# Autodesk Inventor assembly: ProbeHead V3 - Assembly
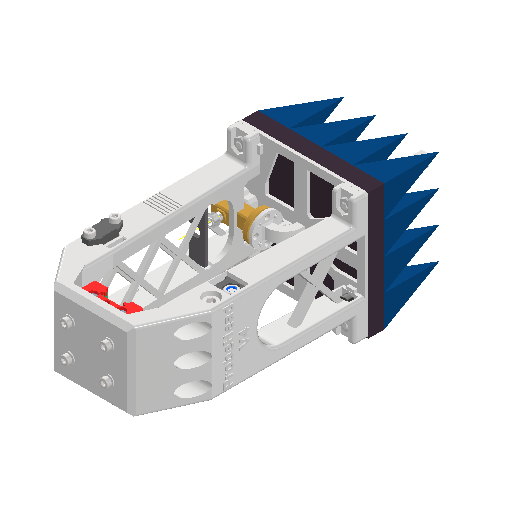
[picture p0: Inventor's stored thumbnail of the model, 512x512]
Saved by Autodesk Inventor 2023.2 (Build 272271000, 271)
## iProperties
Created: 2024-02-09
Part Number: ProbeHead V3 - Assembly
Document SubType Name: Assembly
Designer: Nils Bade
Author: Nils Bade
## Documents named in this file (17)
- C:\Users\nilsb\Documents\Inventor\Projektarbeit-Bade\RatRig_modified\ProbeHead\ProbeHead V4 - Assembly.iam
- C:\Users\nilsb\Documents\Inventor\Projektarbeit-Bade\RatRig_modified\MGN15 Linear-Rail-Block.ipt
- C:\Users\nilsb\Documents\Inventor\Projektarbeit-Bade\RatRig_Standards\face_belt_grabber v2.ipt
- C:\Users\nilsb\Documents\Inventor\Projektarbeit-Bade\Schrauben\Cap Head Screw M3x12 v2.ipt
- C:\Users\nilsb\Documents\Inventor\Projektarbeit-Bade\RatRig_Standards\Hex Nut - M3 v2.ipt
- C:\Users\nilsb\Documents\Inventor\Projektarbeit-Bade\Schrauben\Cap Head Screw M5x40 v2.ipt
- C:\Users\nilsb\Documents\Inventor\Projektarbeit-Bade\RatRig_Standards\Hex Locking Nut - M5 v2.ipt
- C:\Users\nilsb\Documents\Inventor\Projektarbeit-Bade\Schrauben\Washer Simple M3 - DIN6902.ipt
- C:\Users\nilsb\Documents\Inventor\Projektarbeit-Bade\RatRig_modified\ProbeHead\Wire2Probe_Eravant_SWC-15VF-R1-V.ipt
- C:\Users\nilsb\Documents\Inventor\Projektarbeit-Bade\Enclosure\Absorber\Absorber - IHF-Mini.ipt
- C:\Users\nilsb\Documents\Inventor\Projektarbeit-Bade\RatRig_modified\core_xy_belt_grabber_Bade.ipt
- C:\Users\nilsb\Documents\Inventor\Projektarbeit-Bade\RatRig_modified\ProbeHead\ProbeHead_Kabelfixieung_V1.ipt
- C:\Users\nilsb\Documents\Inventor\Projektarbeit-Bade\Enclosure\Magnet-RatrigEnclosure.ipt
- C:\Users\nilsb\Documents\Inventor\Projektarbeit-Bade\RatRig_Standards\Hex Nut - M4 DIN934.ipt
- C:\Users\nilsb\Documents\Inventor\Projektarbeit-Bade\Schrauben\Cap Head Screw M4x8 - DIN912.ipt
- C:\Users\nilsb\Documents\Inventor\Projektarbeit-Bade\RatRig_modified\ProbeHead\ProbeHead-Arms V4.ipt
- C:\Users\nilsb\Documents\Inventor\Projektarbeit-Bade\RatRig_modified\ProbeHead\ProbeAntennas\ProbeAntenna_V1_Long.ipt
## Components (58 placed, 16 different names)
1. ProbeHead-Arms_V4:1 — Passend:96, Passend:97
2. core_xy_belt_grabber_Bade:2
3. core_xy_belt_grabber_Bade:1
4. MGN15 Linear-Rail-Block:1
5. face_belt_grabber v2:1 — Passend:16, Passend:17, Passend:18, Passend:19
6. face_belt_grabber v2:2 — Passend:12, Passend:13, Passend:14, Passend:15
7. Cap Head Screw M3x12 v2:1 — Passend:16, Passend:18, Passend:20
8. Cap Head Screw M3x12 v2:2 — Passend:17, Passend:19, Passend:21
9. Cap Head Screw M3x12 v2:3 — Passend:12, Passend:14, Passend:22
10. Cap Head Screw M3x12 v2:4 — Passend:13, Passend:15, Passend:23
11. Hex Nut - M3 v2:1 — Passend:20
12. Hex Nut - M3 v2:2 — Passend:23
13. Hex Nut - M3 v2:3 — Passend:22
14. Hex Nut - M3 v2:4 — Passend:21
15. Cap Head Screw M5x40 v2:1 — Passend:34
16. Cap Head Screw M5x40 v2:2
17. Hex Locking Nut - M5 v2:1
18. Hex Locking Nut - M5 v2:2 — Passend:34
19. Washer Simple M3 - DIN6902:1 — Passend:59
20. Washer Simple M3 - DIN6902:2 — Passend:56
21. Washer Simple M3 - DIN6902:3 — Passend:58
22. Washer Simple M3 - DIN6902:4 — Passend:57
23. Cap Head Screw M3x12 v2:5 — Passend:59
24. Cap Head Screw M3x12 v2:6 — Passend:58
25. Cap Head Screw M3x12 v2:7 — Passend:56
26. Cap Head Screw M3x12 v2:8 — Passend:57
27. Wire2Probe_Eravant_SWC-15VF-R1-V:1 — Passend:68
28. ProbeAntenna V1 Long:1
29. ProbeHead_Kabelfixieung_V1:1 — Passend:68
30. Magnet-RatrigEnclosure:1
31. Magnet-RatrigEnclosure:2
32. Magnet-RatrigEnclosure:3
33. Magnet-RatrigEnclosure:4
34. Magnet-RatrigEnclosure:5
35. Hex Nut - M4 DIN934:1 — Passend:101
36. Hex Nut - M4 DIN934:2 — Passend:98
37. Hex Nut - M4 DIN934:3 — Passend:99
38. Hex Nut - M4 DIN934:4 — Passend:100
39. Cap Head Screw M4x8 - DIN912:1 — Passend:99
40. Cap Head Screw M4x8 - DIN912:2 — Passend:97, Passend:98
41. Cap Head Screw M4x8 - DIN912:3 — Passend:101
42. Cap Head Screw M4x8 - DIN912:4 — Passend:96, Passend:100
43. Absorber - IHF-Mini:1
44. Absorber - IHF-Mini:18
45. Absorber - IHF-Mini:19
46. Absorber - IHF-Mini:4
47. Absorber - IHF-Mini:22
48. Absorber - IHF-Mini:21
49. Absorber - IHF-Mini:7
50. Absorber - IHF-Mini:8
51. Absorber - IHF-Mini:23
52. Absorber - IHF-Mini:24
53. Absorber - IHF-Mini:11
54. Absorber - IHF-Mini:17
55. Absorber - IHF-Mini:25
56. Absorber - IHF-Mini:26
57. Absorber - IHF-Mini:27
58. Absorber - IHF-Mini:16
## Component patterns: (16 elements, first: Absorber - IHF-Mini:1)
## Relationships (102: Mate 85, Angle 13, Flush 4)
- [Mate]: ProbeHead-Arms_V4:1 ↔ MGN15 Linear-Rail-Block:1
- [Mate]: ProbeHead-Arms_V4:1 ↔ MGN15 Linear-Rail-Block:1
- [Mate]: ProbeHead-Arms_V4:1 ↔ MGN15 Linear-Rail-Block:1
- [Mate]: ProbeHead-Arms_V4:1 ↔ core_xy_belt_grabber_Bade:1
- [Angle] (0 deg): ProbeHead-Arms_V4:1 ↔ core_xy_belt_grabber_Bade:2
- [Mate]: ProbeHead-Arms_V4:1 ↔ core_xy_belt_grabber_Bade:2
- [Flush] (2 mm): ProbeHead-Arms_V4:1 ↔ core_xy_belt_grabber_Bade:2
- [Flush] (2 mm): ProbeHead-Arms_V4:1 ↔ core_xy_belt_grabber_Bade:1
- [Mate]: ProbeHead-Arms_V4:1 ↔ face_belt_grabber v2:2
- [Mate]: ProbeHead-Arms_V4:1 ↔ face_belt_grabber v2:2
- [Mate]: ProbeHead-Arms_V4:1 ↔ face_belt_grabber v2:1
- [Mate]: ProbeHead-Arms_V4:1 ↔ face_belt_grabber v2:1
- Passend:12 [Mate]: face_belt_grabber v2:2 ↔ Cap Head Screw M3x12 v2:3
- Passend:13 [Mate]: face_belt_grabber v2:2 ↔ Cap Head Screw M3x12 v2:4
- Passend:14 [Mate]: face_belt_grabber v2:2 ↔ Cap Head Screw M3x12 v2:3
- Passend:15 [Mate]: face_belt_grabber v2:2 ↔ Cap Head Screw M3x12 v2:4
- Passend:16 [Mate]: face_belt_grabber v2:1 ↔ Cap Head Screw M3x12 v2:1
- Passend:17 [Mate]: face_belt_grabber v2:1 ↔ Cap Head Screw M3x12 v2:2
- Passend:18 [Mate]: face_belt_grabber v2:1 ↔ Cap Head Screw M3x12 v2:1
- Passend:19 [Mate]: face_belt_grabber v2:1 ↔ Cap Head Screw M3x12 v2:2
- Passend:20 [Mate]: Cap Head Screw M3x12 v2:1 ↔ Hex Nut - M3 v2:1
- Passend:21 [Mate]: Cap Head Screw M3x12 v2:2 ↔ Hex Nut - M3 v2:4
- Passend:22 [Mate]: Cap Head Screw M3x12 v2:3 ↔ Hex Nut - M3 v2:3
- Passend:23 [Mate]: Cap Head Screw M3x12 v2:4 ↔ Hex Nut - M3 v2:2
- [Angle] (0 deg): ProbeHead-Arms_V4:1 ↔ Hex Nut - M3 v2:1
- [Angle] (0 deg): ProbeHead-Arms_V4:1 ↔ Hex Nut - M3 v2:3
- [Mate]: ProbeHead-Arms_V4:1 ↔ Hex Nut - M3 v2:3
- [Mate]: ProbeHead-Arms_V4:1 ↔ Hex Nut - M3 v2:2
- [Mate]: ProbeHead-Arms_V4:1 ↔ Hex Nut - M3 v2:1
- [Mate]: ProbeHead-Arms_V4:1 ↔ Hex Nut - M3 v2:4
- [Mate]: ProbeHead-Arms_V4:1 ↔ Cap Head Screw M5x40 v2:2
- [Mate]: ProbeHead-Arms_V4:1 ↔ Cap Head Screw M5x40 v2:1
- [Mate]: ProbeHead-Arms_V4:1 ↔ Cap Head Screw M5x40 v2:1
- [Mate]: ProbeHead-Arms_V4:1 ↔ Cap Head Screw M5x40 v2:2
- [Mate]: core_xy_belt_grabber_Bade:1 ↔ Hex Locking Nut - M5 v2:1
- [Mate]: core_xy_belt_grabber_Bade:1 ↔ Hex Locking Nut - M5 v2:1
- Passend:34 [Mate]: Cap Head Screw M5x40 v2:1 ↔ Hex Locking Nut - M5 v2:2
- [Angle] (0 deg): core_xy_belt_grabber_Bade:2 ↔ Hex Locking Nut - M5 v2:2
- [Mate]: core_xy_belt_grabber_Bade:2 ↔ Hex Locking Nut - M5 v2:2
- [Angle] (0 deg): core_xy_belt_grabber_Bade:1 ↔ Hex Locking Nut - M5 v2:1
- [Mate]: ProbeHead-Arms_V4:1 ↔ Washer Simple M3 - DIN6902:1
- [Mate]: ProbeHead-Arms_V4:1 ↔ Washer Simple M3 - DIN6902:2
- [Mate]: ProbeHead-Arms_V4:1 ↔ Washer Simple M3 - DIN6902:3
- [Mate]: ProbeHead-Arms_V4:1 ↔ Washer Simple M3 - DIN6902:4
- [Mate]: ProbeHead-Arms_V4:1 ↔ Washer Simple M3 - DIN6902:4
- [Mate]: ProbeHead-Arms_V4:1 ↔ Washer Simple M3 - DIN6902:2
- [Mate]: ProbeHead-Arms_V4:1 ↔ Washer Simple M3 - DIN6902:1
- [Mate]: ProbeHead-Arms_V4:1 ↔ Washer Simple M3 - DIN6902:3
- [Mate]: ProbeHead-Arms_V4:1 ↔ Cap Head Screw M3x12 v2:5
- [Mate]: ProbeHead-Arms_V4:1 ↔ Cap Head Screw M3x12 v2:6
- [Mate]: ProbeHead-Arms_V4:1 ↔ Cap Head Screw M3x12 v2:7
- [Mate]: ProbeHead-Arms_V4:1 ↔ Cap Head Screw M3x12 v2:8
- Passend:56 [Mate]: Washer Simple M3 - DIN6902:2 ↔ Cap Head Screw M3x12 v2:7
- Passend:57 [Mate]: Washer Simple M3 - DIN6902:4 ↔ Cap Head Screw M3x12 v2:8
- Passend:58 [Mate]: Washer Simple M3 - DIN6902:3 ↔ Cap Head Screw M3x12 v2:6
- Passend:59 [Mate]: Washer Simple M3 - DIN6902:1 ↔ Cap Head Screw M3x12 v2:5
- [Mate]: ProbeHead-Arms_V4:1 ↔ Cap Head Screw M3x12 v2:4
- [Mate]: ProbeHead-Arms_V4:1 ↔ Cap Head Screw M3x12 v2:2
- [Angle] (0 deg): ProbeHead-Arms_V4:1 ↔ Hex Nut - M3 v2:2
- [Angle] (0 deg): ProbeHead-Arms_V4:1 ↔ Hex Nut - M3 v2:4
- [Angle] (180 deg): ProbeHead-Arms_V4:1 ↔ core_xy_belt_grabber_Bade:1
- [Mate]: ProbeHead-Arms_V4:1 ↔ ProbeAntenna V1 Long:1
- [Mate]: Wire2Probe_Eravant_SWC-15VF-R1-V:1 ↔ ProbeAntenna V1 Long:1
- [Angle] (180 deg): Wire2Probe_Eravant_SWC-15VF-R1-V:1 ↔ ProbeAntenna V1 Long:1
- [Mate]: Wire2Probe_Eravant_SWC-15VF-R1-V:1 ↔ ProbeAntenna V1 Long:1
- [Mate]: ProbeHead-Arms_V4:1 ↔ ProbeHead_Kabelfixieung_V1:1
- Passend:68 [Mate]: Wire2Probe_Eravant_SWC-15VF-R1-V:1 ↔ ProbeHead_Kabelfixieung_V1:1
- [Flush]: ProbeAntenna V1 Long:1 ↔ Absorber - IHF-Mini:1
- [Flush]: ProbeAntenna V1 Long:1 ↔ Absorber - IHF-Mini:1
- [Mate]: ProbeAntenna V1 Long:1 ↔ Absorber - IHF-Mini:1
- [Mate]: ProbeHead-Arms_V4:1 ↔ Magnet-RatrigEnclosure:1
- [Mate]: ProbeHead-Arms_V4:1 ↔ Magnet-RatrigEnclosure:4
- [Mate]: ProbeHead-Arms_V4:1 ↔ Magnet-RatrigEnclosure:3
- [Mate]: ProbeHead-Arms_V4:1 ↔ Magnet-RatrigEnclosure:2
- [Mate]: ProbeHead-Arms_V4:1 ↔ Magnet-RatrigEnclosure:4
- [Mate]: ProbeHead-Arms_V4:1 ↔ Magnet-RatrigEnclosure:1
- [Mate]: ProbeHead-Arms_V4:1 ↔ Magnet-RatrigEnclosure:2
- [Mate]: ProbeHead-Arms_V4:1 ↔ Magnet-RatrigEnclosure:3
- [Mate]: ProbeHead-Arms_V4:1 ↔ Magnet-RatrigEnclosure:5
- [Mate]: ProbeHead-Arms_V4:1 ↔ Magnet-RatrigEnclosure:5
- [Angle] (0 deg): ProbeHead-Arms_V4:1 ↔ Hex Nut - M4 DIN934:1
- [Angle] (0 deg): ProbeHead-Arms_V4:1 ↔ Hex Nut - M4 DIN934:2
- [Angle] (0 deg): ProbeHead-Arms_V4:1 ↔ Hex Nut - M4 DIN934:3
- [Angle] (0 deg): ProbeHead-Arms_V4:1 ↔ Hex Nut - M4 DIN934:4
- [Mate]: ProbeHead-Arms_V4:1 ↔ Hex Nut - M4 DIN934:4
- [Mate]: ProbeHead-Arms_V4:1 ↔ Hex Nut - M4 DIN934:3
- [Mate]: ProbeHead-Arms_V4:1 ↔ Hex Nut - M4 DIN934:2
- [Mate]: ProbeHead-Arms_V4:1 ↔ Hex Nut - M4 DIN934:1
- [Mate]: ProbeAntenna V1 Long:1 ↔ Cap Head Screw M4x8 - DIN912:2
- [Mate]: ProbeAntenna V1 Long:1 ↔ Cap Head Screw M4x8 - DIN912:1
- [Mate]: ProbeAntenna V1 Long:1 ↔ Cap Head Screw M4x8 - DIN912:4
- [Mate]: ProbeAntenna V1 Long:1 ↔ Cap Head Screw M4x8 - DIN912:3
- [Mate]: ProbeAntenna V1 Long:1 ↔ Cap Head Screw M4x8 - DIN912:4
- [Mate]: ProbeAntenna V1 Long:1 ↔ Cap Head Screw M4x8 - DIN912:1
- [Mate]: ProbeAntenna V1 Long:1 ↔ Cap Head Screw M4x8 - DIN912:2
- [Mate]: ProbeAntenna V1 Long:1 ↔ Cap Head Screw M4x8 - DIN912:3
- Passend:96 [Mate]: ProbeHead-Arms_V4:1 ↔ Cap Head Screw M4x8 - DIN912:4
- Passend:97 [Mate]: ProbeHead-Arms_V4:1 ↔ Cap Head Screw M4x8 - DIN912:2
- Passend:98 [Mate]: Hex Nut - M4 DIN934:2 ↔ Cap Head Screw M4x8 - DIN912:2
- Passend:99 [Mate]: Hex Nut - M4 DIN934:3 ↔ Cap Head Screw M4x8 - DIN912:1
- Passend:100 [Mate]: Hex Nut - M4 DIN934:4 ↔ Cap Head Screw M4x8 - DIN912:4
- Passend:101 [Mate]: Hex Nut - M4 DIN934:1 ↔ Cap Head Screw M4x8 - DIN912:3
